# Autodesk Inventor assembly: Assembly2
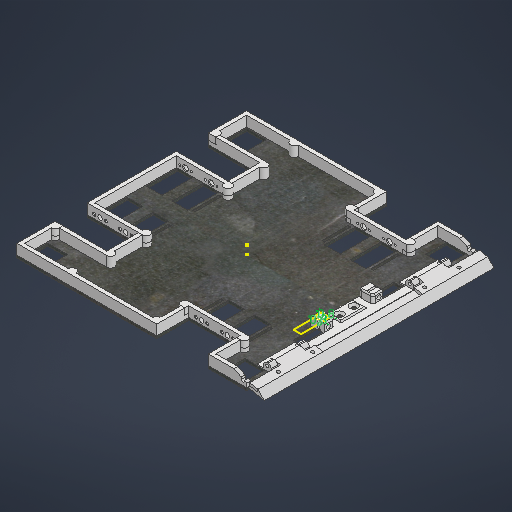
[picture p0: Inventor's stored thumbnail of the model, 512x512]
Saved by Autodesk Inventor 2026.2 (Build 302298010, 298A)
## iProperties
Created: 2026-09-07
Part Number: Assembly2
Document SubType Name: Assembly
Designer: karol
Author: karol
## Documents named in this file (13)
- C:\Users\karol\OneDrive\Dokumenty\GitHub\bolt_v2\ bolt_v2\CAD\Assemblys\mainassembly2.iam
- C:\Users\karol\OneDrive\Dokumenty\GitHub\bolt_v2\ bolt_v2\CAD\ready parts\base2.ipt
- C:\Users\karol\OneDrive\Dokumenty\GitHub\bolt_v2\ bolt_v2\CAD\ready parts\bmw2.ipt
- C:\Users\karol\OneDrive\Dokumenty\GitHub\bolt_v2\ bolt_v2\CAD\ready parts\left\leftbmw2.ipt
- C:\Users\karol\OneDrive\Dokumenty\GitHub\bolt_v2\ bolt_v2\CAD\ready parts\right\rightbmw.ipt
- C:\Users\karol\OneDrive\Dokumenty\GitHub\bolt_v2\ bolt_v2\CAD\ready parts\left\leftwall2.ipt
- C:\Users\karol\OneDrive\Dokumenty\GitHub\bolt_v2\ bolt_v2\CAD\ready parts\right\rightwall2.ipt
- C:\Users\karol\OneDrive\Dokumenty\GitHub\bolt_v2\ bolt_v2\CAD\ready parts\left\leftfrontmotorwall.ipt
- C:\Users\karol\OneDrive\Dokumenty\GitHub\bolt_v2\ bolt_v2\CAD\ready parts\right\rightfrontmotorwall.ipt
- C:\Users\karol\OneDrive\Dokumenty\GitHub\bolt_v2\ bolt_v2\CAD\ready parts\left\leftfrontwall.ipt
- C:\Users\karol\OneDrive\Dokumenty\GitHub\bolt_v2\ bolt_v2\CAD\ready parts\right\rightfrontwall.ipt
- C:\Users\karol\OneDrive\Dokumenty\GitHub\bolt_v2\ bolt_v2\CAD\ready parts\plugassholder.ipt
- C:\Users\karol\OneDrive\Dokumenty\GitHub\bolt_v2\ bolt_v2\CAD\Assemblys\plugassembly2.iam
## Components (12 placed, 12 different names)
1. base2:1 — Flush:1, Flush:2, Flush:3, Flush:4, Flush:5, Flush:6, Flush:7, Flush:8, Flush:9, Flush:10, Flush:11, Flush:12, Flush:13, Flush:14, Flush:15, Flush:16, Flush:17, Flush:18, Mate:1, Mate:2
2. bmw2:1 — Flush:5, Flush:6, Mate:7, Mate:8
3. leftbmw2:1 — Flush:3, Flush:4, Mate:6, Mate:7
4. rightbmw:1 — Flush:7, Flush:8, Mate:8
5. leftwall2:1 — Flush:1, Flush:2, Mate:5, Mate:6
6. rightwall2:1 — Flush:9, Flush:10, Mate:4
7. leftfrontmotorwall:1 — Flush:15, Flush:16, Mate:1, Mate:5
8. rightfrontmotorwall:1 — Flush:13, Flush:14, Mate:3, Mate:4
9. leftfrontwall:1 — Flush:17, Flush:18
10. rightfrontwall:1 — Flush:11, Flush:12, Mate:2, Mate:3
11. plugassholder:1 — Mate:9, Mate:10
12. plugassembly2:1 [sub-assembly] — Mate:9, Mate:10
## Relationships (28: Flush 18, Mate 10)
- Flush:1: base2:1 ↔ leftwall2:1
- Flush:2: base2:1 ↔ leftwall2:1
- Flush:3: base2:1 ↔ leftbmw2:1
- Flush:4: base2:1 ↔ leftbmw2:1
- Flush:5: base2:1 ↔ bmw2:1
- Flush:6: base2:1 ↔ bmw2:1
- Flush:7: base2:1 ↔ rightbmw:1
- Flush:8: base2:1 ↔ rightbmw:1
- Flush:9: base2:1 ↔ rightwall2:1
- Flush:10: base2:1 ↔ rightwall2:1
- Flush:11: base2:1 ↔ rightfrontwall:1
- Flush:12: base2:1 ↔ rightfrontwall:1
- Flush:13: base2:1 ↔ rightfrontmotorwall:1
- Flush:14: base2:1 ↔ rightfrontmotorwall:1
- Flush:15: base2:1 ↔ leftfrontmotorwall:1
- Flush:16: base2:1 ↔ leftfrontmotorwall:1
- Flush:17: base2:1 ↔ leftfrontwall:1
- Flush:18: base2:1 ↔ leftfrontwall:1
- Mate:1: base2:1 ↔ leftfrontmotorwall:1
- Mate:2: base2:1 ↔ rightfrontwall:1
- Mate:3: rightfrontmotorwall:1 ↔ rightfrontwall:1
- Mate:4: rightwall2:1 ↔ rightfrontmotorwall:1
- Mate:5: leftwall2:1 ↔ leftfrontmotorwall:1
- Mate:6: leftbmw2:1 ↔ leftwall2:1
- Mate:7: bmw2:1 ↔ leftbmw2:1
- Mate:8: bmw2:1 ↔ rightbmw:1
- Mate:9: plugassholder:1 ↔ plugassembly2:1
- Mate:10 (0.2 mm): plugassholder:1 ↔ plugassembly2:1
